# Autodesk Inventor assembly: am-0420 8in Rubber Treaded Wheel,iam
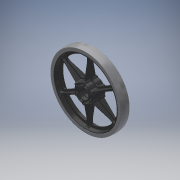
[picture p0: Inventor's stored thumbnail of the model, 180x180]
Saved by Autodesk Inventor 2019 (Build 230136000, 136)
## iProperties
Created: 2019-01-30
Part Number: am-0420 8in Rubber Treaded Wheel,iam
Document SubType Name: Assembly
Designer: Michael Olukoya
Author: Michael Olukoya
## Documents named in this file (3)
- C:\Users\Michael Olukoya\Desktop\Turtle BOT- AI\New Bot components\am-0420 8in Rubber Treaded Wheel.iam
- C:\Users\Michael Olukoya\Desktop\Turtle BOT- AI\New Bot components\8in 2010 FIRST Hub-1-solid1.ipt
- C:\Users\Michael Olukoya\Desktop\Turtle BOT- AI\New Bot components\8in 2010 FIRST Tread-1-solid1.ipt
## Components (2 placed, 2 different names)
1. 8in 2010 FIRST Hub-1-solid1:1 — Flush:1, Rotational:1
2. 8in 2010 FIRST Tread-1-solid1:1 — Flush:1, Rotational:1
## Relationships (2: Flush 1, RevoluteJoint 1)
- Flush:1: 8in 2010 FIRST Hub-1-solid1:1 ↔ 8in 2010 FIRST Tread-1-solid1:1
- Rotational:1 [RevoluteJoint]: 8in 2010 FIRST Hub-1-solid1:1 ↔ 8in 2010 FIRST Tread-1-solid1:1
